# Autodesk Inventor assembly: stack_gear
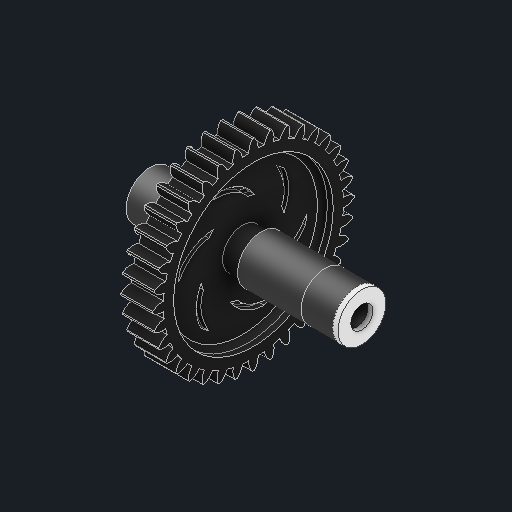
[picture p0: Inventor's stored thumbnail of the model, 512x512]
Saved by Autodesk Inventor 2025 (Build 290162000, 162)
## iProperties
Created: 2024-10-03
Part Number: stack_gear
Document SubType Name: Assembly
Designer: Averey Ku
Author: Averey Ku
## Documents named in this file (8)
- D:\vex_robotics_high_stakes\hardware\cad\bots\high_stakes_v2\chassis\drivebay\stack_gear.iam
- D:\vex_robotics_high_stakes\hardware\cad\robpros_cad_lib\Motion\Gears\LS 36T Gear.ipt
- D:\vex_robotics_high_stakes\hardware\cad\robpros_cad_lib\Motion\Spacers\Spacer Nylon .375 OD\NSpacer .375 OD x .250.ipt
- D:\vex_robotics_high_stakes\hardware\cad\robpros_cad_lib\Motion\Spacers\Spacer Nylon .375 OD.ipt
- D:\vex_robotics_high_stakes\hardware\cad\robpros_cad_lib\Motion\Spacers\Washer Teflon\TWasher .375 OD x .04000.ipt
- D:\vex_robotics_high_stakes\hardware\cad\robpros_cad_lib\Motion\Spacers\Washer Teflon.ipt
- D:\vex_robotics_high_stakes\hardware\cad\robpros_cad_lib\Motion\Spacers\Spacer Nylon .375 OD\NSpacer .375 OD x .500.ipt
- D:\vex_robotics_high_stakes\hardware\cad\robpros_cad_lib\Motion\Shaft LS\Shaft Collar ipts\Shaft Collar Set Screw.ipt
## Components (6 placed, 5 different names)
1. LS 36T Gear:1 — Insert:3, Insert:5
2. NSpacer .375 OD x .250:1 — Insert:2
3. TWasher .375 OD x .04000:1
4. NSpacer .375 OD x .500:2 — Insert:2, Insert:3
5. NSpacer .375 OD x .250:3 — Insert:4
6. Shaft Collar Set Screw:1 — Insert:4, Insert:5
## Relationships (5: Insert 5)
- [Insert]: NSpacer .375 OD x .250:1 ↔ TWasher .375 OD x .04000:1
- Insert:2: NSpacer .375 OD x .250:1 ↔ NSpacer .375 OD x .500:2
- Insert:3: LS 36T Gear:1 ↔ NSpacer .375 OD x .500:2
- Insert:4: NSpacer .375 OD x .250:3 ↔ Shaft Collar Set Screw:1
- Insert:5: LS 36T Gear:1 ↔ Shaft Collar Set Screw:1
